# Autodesk Inventor assembly: 軸フレーム
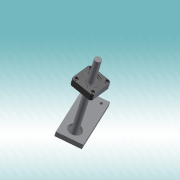
[picture p0: Inventor's stored thumbnail of the model, 180x180]
Saved by Autodesk Inventor 2015 (Build 190159000, 159)
## iProperties
Created: 2016-03-21
Part Number: 軸フレーム
Document SubType Name: Assembly
Designer: buzztaka
Author: buzztaka
## Documents named in this file (10)
- C:\Users\buzztaka\Documents\tukuba\i-cart-middle_3d-model\計測輪アセンブル\軸フレーム.iam
- C:\Users\buzztaka\Documents\tukuba\i-cart-middle_3d-model\計測輪アセンブル\ベアリングホルダ\BGSRB6201ZZ.iam
- C:\Users\buzztaka\Documents\tukuba\i-cart-middle_3d-model\計測輪アセンブル\回転軸取り付け板.ipt
- C:\Users\buzztaka\Documents\tukuba\i-cart-middle_3d-model\計測輪アセンブル\C-SFL6901ZZ.ipt
- C:\Users\buzztaka\Documents\tukuba\i-cart-middle_3d-model\計測輪アセンブル\回転軸.ipt
- C:\Users\buzztaka\Documents\tukuba\i-cart-middle_3d-model\計測輪アセンブル\軸フレーム\AIP\FEA\bq9jranq8.fins
- C:\Users\buzztaka\Documents\tukuba\i-cart-middle_3d-model\計測輪アセンブル\軸フレーム\AIP\FEA\bq9jranr4.fsat
- C:\Users\buzztaka\Documents\tukuba\i-cart-middle_3d-model\計測輪アセンブル\軸フレーム\AIP\FEA\bq9jranr4.ftes
- C:\Users\buzztaka\Documents\tukuba\i-cart-middle_3d-model\計測輪アセンブル\軸フレーム\AIP\FEA\bq9jranr4.fwiz
- C:\Users\buzztaka\Documents\tukuba\i-cart-middle_3d-model\計測輪アセンブル\軸フレーム\AIP\FEA\bq9jranxc.fmsh
## Components (4 placed, 4 different names)
1. 回転軸取り付け板:1
2. C-SFL6901ZZ:1
3. 回転軸:1
4. BGSRB6201ZZ:2 [sub-assembly]
## Relationships (3: Insert 3)
- [Insert]: 回転軸取り付け板:1 ↔ C-SFL6901ZZ:1
- [Insert] (10 mm): C-SFL6901ZZ:1 ↔ 回転軸:1
- [Insert] (-60 mm): 回転軸:1 ↔ BGSRB6201ZZ:2
## Named parameters: d1_d0 = 0 mm, sa_0 = 500
note: some values were not read from the file. Shown as the stored number, unit unknown: "sa_0".
